# Autodesk Inventor assembly: Pedal Assembly
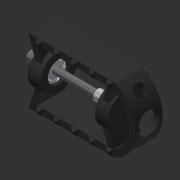
[picture p0: Inventor's stored thumbnail of the model, 180x180]
Saved by Autodesk Inventor 2019 (Build 230136000, 136)
## iProperties
Created: 2020-06-01
Part Number: Pedal Assembly
Document SubType Name: Assembly
Designer: 18186
Author: 18186
## Documents named in this file (6)
- C:\Users\18186\Desktop\Important Shit\Michael Goldberg Portfolio\CAD Portfolio\IPT Files\Bike\Pedal Assembly Right.iam
- C:\Users\18186\Desktop\Important Shit\Michael Goldberg Portfolio\CAD Portfolio\IPT Files\Bike\Pedal.ipt
- C:\Users\18186\Desktop\Important Shit\Michael Goldberg Portfolio\CAD Portfolio\IPT Files\Bike\Bearing.ipt
- C:\Users\18186\Desktop\Important Shit\Michael Goldberg Portfolio\CAD Portfolio\IPT Files\Bike\Pedal Female Right.ipt
- C:\Users\18186\Desktop\Important Shit\Michael Goldberg Portfolio\CAD Portfolio\IPT Files\Bike\Pedal Connector Right.ipt
- C:\Users\18186\Desktop\Important Shit\Michael Goldberg Portfolio\CAD Portfolio\IPT Files\Bike\Pedal Bolt Right.ipt
## Components (6 placed, 5 different names)
1. Pedal:1 — Mate:1, Flush:1, Mate:2, Flush:2, Mate:4
2. Bearing:1 — Mate:2, Flush:2, Mate:5, Flush:3
3. Bearing:2 — Mate:1, Flush:1, Mate:3
4. Pedal Female Right:1 — Mate:3, Mate:4
5. Pedal Connector Right:1 — Mate:5, Flush:3, Mate:6, Flush:4
6. Pedal Bolt Right:1 — Mate:6, Flush:4
## Relationships (10: Mate 6, Flush 4)
- Mate:1: Pedal:1 ↔ Bearing:2
- Flush:1: Pedal:1 ↔ Bearing:2
- Mate:2: Pedal:1 ↔ Bearing:1
- Flush:2: Pedal:1 ↔ Bearing:1
- Mate:3: Bearing:2 ↔ Pedal Female Right:1
- Mate:4: Pedal:1 ↔ Pedal Female Right:1
- Mate:5: Bearing:1 ↔ Pedal Connector Right:1
- Flush:3: Bearing:1 ↔ Pedal Connector Right:1
- Mate:6: Pedal Connector Right:1 ↔ Pedal Bolt Right:1
- Flush:4: Pedal Connector Right:1 ↔ Pedal Bolt Right:1
